# Autodesk Inventor assembly: hdm assemble
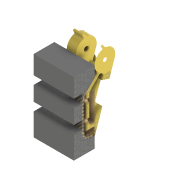
[picture p0: Inventor's stored thumbnail of the model, 180x180]
Saved by Autodesk Inventor 2021 (Build 250183000, 183)
## iProperties
Created: 2022-10-19
Part Number: hdm assemble
Document SubType Name: Assembly
Designer: alyn649
Author: alyn649
## Documents named in this file (4)
- \\files.auckland.ac.nz\myhome\Documents\GitHub\hand\PRINTS\hdm assemble.iam
- \\files.auckland.ac.nz\myhome\Documents\GitHub\hand\HDM\Mould_tip_v2.ipt
- \\files.auckland.ac.nz\myhome\Documents\GitHub\hand\PLANGE7\Phalalnge7_35mm_TIP_hdm.ipt
- \\files.auckland.ac.nz\myhome\Documents\GitHub\hand\HDM_represent\flange7-tip.ipt
## Components (3 placed, 3 different names)
1. Mould_tip_v2:1 — Planar:1, Mate:1, Mate:2, Angle:1
2. Phalalnge7_35mm_TIP_hdm:1 — Planar:1, Mate:1, Mate:2, Mate:3, Rigid:1
3. flange7-tip:1 — Rigid:1
## Relationships (6: Mate 3, PlanarJoint 1, Angle 1, WeldJoint 1)
- Planar:1: Mould_tip_v2:1 ↔ Phalalnge7_35mm_TIP_hdm:1
- Mate:1: Mould_tip_v2:1 ↔ Phalalnge7_35mm_TIP_hdm:1
- Mate:2: Mould_tip_v2:1 ↔ Phalalnge7_35mm_TIP_hdm:1
- Mate:3: Phalalnge7_35mm_TIP_hdm:1
- Angle:1 (0 deg): Mould_tip_v2:1
- Rigid:1 [WeldJoint]: Phalalnge7_35mm_TIP_hdm:1 ↔ flange7-tip:1
